# Autodesk Inventor assembly: assembled-feed_feedline_8in
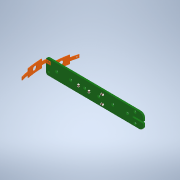
[picture p0: Inventor's stored thumbnail of the model, 180x180]
Saved by Autodesk Inventor 2021 (Build 250183000, 183)
## iProperties
Created: 2020-10-06
Part Number: assembled-feed_feedline_8in
Document SubType Name: Assembly
Designer: dsouthall
Author: dsouthall
## iProperties of the stored document tri-slot-feedlines.iam
Company: A Company
Created: 2020-10-06
Part Number: tri-slot-feedlines
Description: KiCad electronic assembly
Document SubType Name: Assembly
Designer: dsouthall
Authority: Unknown
Sending System: KiCad to STEP converter
Preprocessor: Open CASCADE STEP processor 6.9
Title: tri-slot-feedlines.step
Author: An Author
## iProperties of the stored document C_0805_2012Metric.iam
Created: 2020-10-06
Part Number: C_0805_2012Metric
Document SubType Name: Assembly
Designer: dsouthall
Author: dsouthall
## iProperties of the stored document TestPoint_Loop_D3.80mm_Drill2.0mm.iam
Created: 2020-10-06
Part Number: TestPoint_Loop_D3.80mm_Drill2.0mm
Document SubType Name: Assembly
Designer: dsouthall
Author: dsouthall
## iProperties of the stored document SOLID.ipt
Created: 2020-10-06
Part Number: SOLID
Material: Generic
Document SubType Name: Modeling
Designer: dsouthall
Density: 1 g/cm^3
Appearance: Default
Author: dsouthall
## iProperties of the stored document SOLID_1.ipt
Created: 2020-10-06
Part Number: SOLID_1
Material: Generic
Document SubType Name: Modeling
Designer: dsouthall
Density: 1 g/cm^3
Appearance: Default
Author: dsouthall
## iProperties of the stored document COMPOUND.ipt
Created: 2020-10-06
Part Number: COMPOUND
Material: Generic
Document SubType Name: Modeling
Designer: dsouthall
Density: 1 g/cm^3
Appearance: Default
Author: dsouthall
## Documents named in this file (11)
- C:\Users\dsouthall\OneDrive - The University of Chicago\Hpol\Model 8 in\assembled-feed_feedline_8in.iam
- **C:\Users\dsouthall\OneDrive - The University of Chicago\Hpol\Model 8 in\assembled-feed_feedline_8in.iam*LocalDocs*xAaaaaedaAaaaaaaaAaaaqzqe3f*tri-slot-feedlines.iam
- C:\Users\dsouthall\OneDrive - The University of Chicago\Hpol\Model 8 in\source\digikey-mockup-A114140-ND.ipt
- **C:\Users\dsouthall\OneDrive - The University of Chicago\Hpol\Model 8 in\assembled-feed_feedline_8in.iam*LocalDocs*xAaaaabbaAaaaaaaaAaaaq43cWb*C_0805_2012Metric.iam
- **C:\Users\dsouthall\OneDrive - The University of Chicago\Hpol\Model 8 in\assembled-feed_feedline_8in.iam*LocalDocs*xAaaaqeaaAaaaaaaaAaaaqpa5Wa*TestPoint_Loop_D3.80mm_Drill2.0mm.iam
- **C:\Users\dsouthall\OneDrive - The University of Chicago\Hpol\Model 8 in\assembled-feed_feedline_8in.iam*LocalDocs*xAaaaqkbaAaaaaaaaAaaaqmw0Yh*COMPOUND.ipt
- **C:\Users\dsouthall\OneDrive - The University of Chicago\Hpol\Model\assembled-feed_feedline_8in.iam*LocalDocs*xAaaaabbaAaaaaaaaAaaaq43cWb*C_0805_2012Metric.iam
- **C:\Users\dsouthall\OneDrive - The University of Chicago\Hpol\Model\assembled-feed_feedline_8in.iam*LocalDocs*xAaaaqcaaAaaaaaaaAaaaquciMe*SOLID.ipt
- **C:\Users\dsouthall\OneDrive - The University of Chicago\Hpol\Model 8 in\assembled-feed_feedline_8in.iam*LocalDocs*xAaaaqebaAaaaaaaaAaaaaurr4a*SOLID_1.ipt
- **C:\Users\dsouthall\OneDrive - The University of Chicago\Hpol\Model\assembled-feed_feedline_8in.iam*LocalDocs*xAaaaqebaAaaaaaaaAaaaaurr4a*SOLID_1.ipt
- C:\Users\dsouthall\OneDrive - The University of Chicago\Hpol\Feed Design\tri-slot-feedlines_revC\tri-slot-feedlines.step
## Components (3 placed, 2 different names)
1. tri-slot-feedlines:1 [sub-assembly] — Angle:1, Insert:2, Angle:2, Insert:3
2. digikey-mockup-A114140-ND:1 — Angle:1, Insert:3
3. digikey-mockup-A114140-ND:2 — Insert:2, Angle:2
## Relationships (4: Angle 2, Insert 2)
- Angle:1 (180 deg): tri-slot-feedlines:1 ↔ digikey-mockup-A114140-ND:1
- Insert:2: tri-slot-feedlines:1 ↔ digikey-mockup-A114140-ND:2
- Angle:2 (0 deg): tri-slot-feedlines:1 ↔ digikey-mockup-A114140-ND:2
- Insert:3: tri-slot-feedlines:1 ↔ digikey-mockup-A114140-ND:1
